# Autodesk Inventor assembly: Conjunto
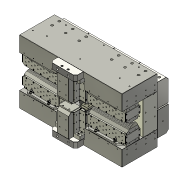
[picture p0: Inventor's stored thumbnail of the model, 180x180]
Saved by Autodesk Inventor 2016 (Build 200138000, 138)
## iProperties
Created: 2015-09-16
Part Number: Conjunto
Document SubType Name: Assembly
Designer: Reinaldo.Basílio
Mass: 1.22159e+06 g
Surface Area: 105771 cm^2
Volume: 178750 cm^3
Density: 6.83406 g/cm^3
Project: DIPOLO BC-3T- SIRIUS
Description: DIPOLO BC-3T- SIRIUS
Cost Center: 1504002005
Author: reinaldo.basilio
Title: DIPOLO BC-3T- SIRIUS
Subject: Conjunto
## Documents named in this file (13)
- R:\LNLS\Grupos\IMA\Sirius\Projetos\SIRIUS-Magnets\Magnets-SI\si-dipoles-bc\Prototipo 1\Projeto Mecanico\BC-100000.iam
- D:\ARQ\Basilio\LNLS-2\Anel\Dipolos\BC-3T\Dipolo 3T e 1T\Prototipo 1\Projeto Mecanico\BC-10010.ipt
- D:\ARQ\Basilio\LNLS-2\Anel\Dipolos\BC-3T\Dipolo 3T e 1T\Prototipo 1\Projeto Mecanico\BC-100000-Inf.iam
- D:\ARQ\Basilio\LNLS-2\Anel\Dipolos\BC-3T\Dipolo 3T e 1T\Prototipo 1\Projeto Mecanico\BC-100000-Sup.iam
- D:\ARQ\Basilio\LNLS-2\Anel\Dipolos\BC-3T\Dipolo 3T e 1T\Prototipo 1\Projeto Mecanico\Parafusos\DIN 912 - M12x110.ipt
- D:\ARQ\Basilio\LNLS-2\Anel\Dipolos\BC-3T\Dipolo 3T e 1T\Prototipo 1\Projeto Mecanico\Parafusos\DIN 912 - M12x120.ipt
- D:\ARQ\Basilio\LNLS-2\Anel\Dipolos\BC-3T\Dipolo 3T e 1T\Prototipo 1\Projeto Mecanico\BC-100001\AIP\FEA\bjj5sjykh.fres
- D:\ARQ\Basilio\LNLS-2\Anel\Dipolos\BC-3T\Dipolo 3T e 1T\Prototipo 1\Projeto Mecanico\BC-100000\AIP\FEA\blkui5reo.fins
- D:\ARQ\Basilio\LNLS-2\Anel\Dipolos\BC-3T\Dipolo 3T e 1T\Prototipo 1\Projeto Mecanico\BC-100000\AIP\FEA\blkui5reo.fsat
- D:\ARQ\Basilio\LNLS-2\Anel\Dipolos\BC-3T\Dipolo 3T e 1T\Prototipo 1\Projeto Mecanico\BC-100000\AIP\FEA\blkui5reo.ftes
- D:\ARQ\Basilio\LNLS-2\Anel\Dipolos\BC-3T\Dipolo 3T e 1T\Prototipo 1\Projeto Mecanico\BC-100000\AIP\FEA\blkui5reo.fwiz
- D:\ARQ\Basilio\LNLS-2\Anel\Dipolos\BC-3T\Dipolo 3T e 1T\Prototipo 1\Projeto Mecanico\BC-100000\AIP\FEA\blkui5s3k.fmsh
- D:\ARQ\Basilio\LNLS-2\Anel\Dipolos\BC-3T\Dipolo 3T e 1T\Prototipo 1\Projeto Mecanico\BC-100000\AIP\FEA\blkui5s3l.fres
## Components (36 placed, 5 different names)
1. BC-100000-Inf:1 [sub-assembly] — Insert:1, Insert:2, Insert:3, Insert:4, Insert:19, Insert:20, Insert:21, Insert:22, Insert:23, Insert:24, Insert:25, Insert:26, Insert:27, Insert:28, Insert:29, Insert:30
2. BC-10010:1 — Insert:1, Insert:4, Insert:5
3. BC-10010:2 — Insert:2, Insert:3, Insert:6
4. BC-100000-Sup:1 [sub-assembly] — Insert:5, Insert:6, Insert:7, Insert:8, Insert:9, Insert:10, Insert:11, Insert:12, Insert:13, Insert:14, Insert:15, Insert:16, Insert:17, Insert:18, Insert:31, Insert:32, Insert:33, Insert:34, Insert:35, Insert:36, Insert:37, Insert:38
5. DIN 912 - Parafuso Allen com cabeça (inox) M12x110:1 — Insert:8
6. DIN 912 - Parafuso Allen com cabeça (inox) M12x110:2 — Insert:7
7. DIN 912 - Parafuso Allen com cabeça (inox) M12x110:3 — Insert:10
8. DIN 912 - Parafuso Allen com cabeça (inox) M12x110:4 — Insert:9
9. DIN 912 - Parafuso Allen com cabeça (inox) M12x110:5 — Insert:12
10. DIN 912 - Parafuso Allen com cabeça (inox) M12x110:6 — Insert:11
11. DIN 912 - Parafuso Allen com cabeça (inox) M12x110:7 — Insert:14
12. DIN 912 - Parafuso Allen com cabeça (inox) M12x110:8 — Insert:13
13. DIN 912 - Parafuso Allen com cabeça (inox) M12x110:9 — Insert:16
14. DIN 912 - Parafuso Allen com cabeça (inox) M12x110:10 — Insert:15
15. DIN 912 - Parafuso Allen com cabeça (inox) M12x110:11 — Insert:18
16. DIN 912 - Parafuso Allen com cabeça (inox) M12x110:12 — Insert:17
17. DIN 912 - Parafuso Allen com cabeça (inox) M12x110:13 — Insert:19
18. DIN 912 - Parafuso Allen com cabeça (inox) M12x110:14 — Insert:20
19. DIN 912 - Parafuso Allen com cabeça (inox) M12x110:15 — Insert:22
20. DIN 912 - Parafuso Allen com cabeça (inox) M12x110:16 — Insert:21
21. DIN 912 - Parafuso Allen com cabeça (inox) M12x110:17 — Insert:24
22. DIN 912 - Parafuso Allen com cabeça (inox) M12x110:18 — Insert:23
23. DIN 912 - Parafuso Allen com cabeça (inox) M12x110:19 — Insert:26
24. DIN 912 - Parafuso Allen com cabeça (inox) M12x110:20 — Insert:25
25. DIN 912 - Parafuso Allen com cabeça (inox) M12x110:21 — Insert:28
26. DIN 912 - Parafuso Allen com cabeça (inox) M12x110:22 — Insert:27
27. DIN 912 - Parafuso Allen com cabeça (inox) M12x110:23 — Insert:30
28. DIN 912 - Parafuso Allen com cabeça (inox) M12x110:24 — Insert:29
29. DIN 912 - Parafuso Allen com cabeça (inox) M12x120:1 — Insert:31
30. DIN 912 - Parafuso Allen com cabeça (inox) M12x120:2 — Insert:32
31. DIN 912 - Parafuso Allen com cabeça (inox) M12x120:3 — Insert:33
32. DIN 912 - Parafuso Allen com cabeça (inox) M12x120:4 — Insert:34
33. DIN 912 - Parafuso Allen com cabeça (inox) M12x120:5 — Insert:35
34. DIN 912 - Parafuso Allen com cabeça (inox) M12x120:6 — Insert:36
35. DIN 912 - Parafuso Allen com cabeça (inox) M12x120:7 — Insert:37
36. DIN 912 - Parafuso Allen com cabeça (inox) M12x120:8 — Insert:38
## Relationships (38: Insert 38)
- Insert:1: BC-100000-Inf:1 ↔ BC-10010:1
- Insert:2: BC-100000-Inf:1 ↔ BC-10010:2
- Insert:3: BC-100000-Inf:1 ↔ BC-10010:2
- Insert:4: BC-100000-Inf:1 ↔ BC-10010:1
- Insert:5: BC-10010:1 ↔ BC-100000-Sup:1
- Insert:6: BC-10010:2 ↔ BC-100000-Sup:1
- Insert:7: BC-100000-Sup:1 ↔ DIN 912 - Parafuso Allen com cabeça (inox) M12x110:2
- Insert:8: BC-100000-Sup:1 ↔ DIN 912 - Parafuso Allen com cabeça (inox) M12x110:1
- Insert:9: BC-100000-Sup:1 ↔ DIN 912 - Parafuso Allen com cabeça (inox) M12x110:4
- Insert:10: BC-100000-Sup:1 ↔ DIN 912 - Parafuso Allen com cabeça (inox) M12x110:3
- Insert:11: BC-100000-Sup:1 ↔ DIN 912 - Parafuso Allen com cabeça (inox) M12x110:6
- Insert:12: BC-100000-Sup:1 ↔ DIN 912 - Parafuso Allen com cabeça (inox) M12x110:5
- Insert:13: BC-100000-Sup:1 ↔ DIN 912 - Parafuso Allen com cabeça (inox) M12x110:8
- Insert:14: BC-100000-Sup:1 ↔ DIN 912 - Parafuso Allen com cabeça (inox) M12x110:7
- Insert:15: BC-100000-Sup:1 ↔ DIN 912 - Parafuso Allen com cabeça (inox) M12x110:10
- Insert:16: BC-100000-Sup:1 ↔ DIN 912 - Parafuso Allen com cabeça (inox) M12x110:9
- Insert:17: BC-100000-Sup:1 ↔ DIN 912 - Parafuso Allen com cabeça (inox) M12x110:12
- Insert:18: BC-100000-Sup:1 ↔ DIN 912 - Parafuso Allen com cabeça (inox) M12x110:11
- Insert:19: BC-100000-Inf:1 ↔ DIN 912 - Parafuso Allen com cabeça (inox) M12x110:13
- Insert:20: BC-100000-Inf:1 ↔ DIN 912 - Parafuso Allen com cabeça (inox) M12x110:14
- Insert:21: BC-100000-Inf:1 ↔ DIN 912 - Parafuso Allen com cabeça (inox) M12x110:16
- Insert:22: BC-100000-Inf:1 ↔ DIN 912 - Parafuso Allen com cabeça (inox) M12x110:15
- Insert:23: BC-100000-Inf:1 ↔ DIN 912 - Parafuso Allen com cabeça (inox) M12x110:18
- Insert:24: BC-100000-Inf:1 ↔ DIN 912 - Parafuso Allen com cabeça (inox) M12x110:17
- Insert:25: BC-100000-Inf:1 ↔ DIN 912 - Parafuso Allen com cabeça (inox) M12x110:20
- Insert:26: BC-100000-Inf:1 ↔ DIN 912 - Parafuso Allen com cabeça (inox) M12x110:19
- Insert:27: BC-100000-Inf:1 ↔ DIN 912 - Parafuso Allen com cabeça (inox) M12x110:22
- Insert:28: BC-100000-Inf:1 ↔ DIN 912 - Parafuso Allen com cabeça (inox) M12x110:21
- Insert:29: BC-100000-Inf:1 ↔ DIN 912 - Parafuso Allen com cabeça (inox) M12x110:24
- Insert:30: BC-100000-Inf:1 ↔ DIN 912 - Parafuso Allen com cabeça (inox) M12x110:23
- Insert:31 (45 mm): BC-100000-Sup:1 ↔ DIN 912 - Parafuso Allen com cabeça (inox) M12x120:1
- Insert:32 (45 mm): BC-100000-Sup:1 ↔ DIN 912 - Parafuso Allen com cabeça (inox) M12x120:2
- Insert:33 (45 mm): BC-100000-Sup:1 ↔ DIN 912 - Parafuso Allen com cabeça (inox) M12x120:3
- Insert:34 (45 mm): BC-100000-Sup:1 ↔ DIN 912 - Parafuso Allen com cabeça (inox) M12x120:4
- Insert:35 (45 mm): BC-100000-Sup:1 ↔ DIN 912 - Parafuso Allen com cabeça (inox) M12x120:5
- Insert:36 (45 mm): BC-100000-Sup:1 ↔ DIN 912 - Parafuso Allen com cabeça (inox) M12x120:6
- Insert:37 (45 mm): BC-100000-Sup:1 ↔ DIN 912 - Parafuso Allen com cabeça (inox) M12x120:7
- Insert:38 (45 mm): BC-100000-Sup:1 ↔ DIN 912 - Parafuso Allen com cabeça (inox) M12x120:8
## Named parameters: sa_0 = -7.2892e-08, sa_1 = -2.04075e-06, sa_2 = -6e+06
note: some values were not read from the file. Shown as the stored number, unit unknown: "sa_0", "sa_1", "sa_2".
